# Autodesk Inventor assembly: Assembly_HCMUTE-CDT23-CB_E3F-DS30C4
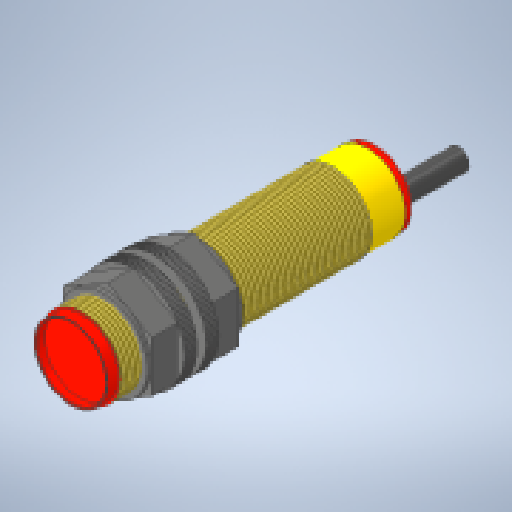
[picture p0: Inventor's stored thumbnail of the model, 512x512]
Saved by Autodesk Inventor 2023 (Build 270158000, 158)
## iProperties
Created: 2023-10-11
Part Number: Assembly_HCMUTE-CDT23-CB_E3F-DS30C4
Document SubType Name: Assembly
Designer: havie
Author: havie
## Documents named in this file (3)
- C:\Users\havie\Desktop\DO_AN_CDT\1.PART\Assembly_HCMUTE-CDT23-CB_E3F-DS30C4.iam
- C:\Users\havie\Desktop\DO_AN_CDT\1.PART\2309HCMUTE-CDT23-CB_CLAMP-NUT.ipt
- C:\Users\havie\Desktop\DO_AN_CDT\1.PART\2309HCMUTE-CDT23-CB_SHAPE.ipt
## Components (3 placed, 2 different names)
1. 2309HCMUTE-CDT23-CB_CLAMP-NUT:1 — Mate:1, Flush:1, Mate:2, Angle:1
2. 2309HCMUTE-CDT23-CB_SHAPE:1 — Mate:1, Flush:1, Mate:3
3. 2309HCMUTE-CDT23-CB_CLAMP-NUT:2 — Mate:2, Mate:3, Angle:1
## Relationships (5: Mate 3, Flush 1, Angle 1)
- Mate:1: 2309HCMUTE-CDT23-CB_CLAMP-NUT:1 ↔ 2309HCMUTE-CDT23-CB_SHAPE:1
- Flush:1 (5 mm): 2309HCMUTE-CDT23-CB_CLAMP-NUT:1 ↔ 2309HCMUTE-CDT23-CB_SHAPE:1
- Mate:2 (2 mm): 2309HCMUTE-CDT23-CB_CLAMP-NUT:1 ↔ 2309HCMUTE-CDT23-CB_CLAMP-NUT:2
- Mate:3: 2309HCMUTE-CDT23-CB_SHAPE:1 ↔ 2309HCMUTE-CDT23-CB_CLAMP-NUT:2
- Angle:1 (0 deg): 2309HCMUTE-CDT23-CB_CLAMP-NUT:1 ↔ 2309HCMUTE-CDT23-CB_CLAMP-NUT:2
